# Autodesk Inventor assembly: Chain Testing 9-16-19
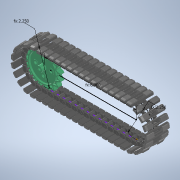
[picture p0: Inventor's stored thumbnail of the model, 180x180]
Saved by Autodesk Inventor 2020 (Build 240168000, 168)
## iProperties
Created: 2019-09-16
Part Number: Chain Testing 9-16-19
Document SubType Name: Assembly
Designer: Corey
Author: Corey
## Documents named in this file (4)
- C:\Users\Corey\Documents\Tower-Takeover-CAD\Chain Testing 9-16-19.iam
- C:\Users\Corey\Documents\Tower-Takeover-CAD\Parts\Motion\Chain & Tank Tread\Tank Tread Traction Link.ipt
- C:\Users\Corey\Documents\Tower-Takeover-CAD\Chain Sketch 9-16-9.ipt
- C:\Users\Corey\Documents\Tower-Takeover-CAD\Parts\Motion\Sprockets\High Strength 18-tooth Sprocket.ipt
## Components (51 placed, 3 different names)
1. Chain Sketch 9-16-9:1 — Flush:1, Flush:2, Flush:3, Flush:4, Flush:5, Flush:6
2. High Strength 18-tooth Sprocket:1 — Flush:4, Flush:5, Flush:6
3. Tank Tread Traction Link:1 — Flush:1, Flush:2, Flush:3
4. Tank Tread Traction Link:2
5. Tank Tread Traction Link:3
6. Tank Tread Traction Link:4
7. Tank Tread Traction Link:5
8. Tank Tread Traction Link:6
9. Tank Tread Traction Link:7
10. Tank Tread Traction Link:8
11. Tank Tread Traction Link:9
12. Tank Tread Traction Link:10
13. Tank Tread Traction Link:11
14. Tank Tread Traction Link:12
15. Tank Tread Traction Link:13
16. Tank Tread Traction Link:14
17. Tank Tread Traction Link:15
18. Tank Tread Traction Link:16
19. Tank Tread Traction Link:17
20. Tank Tread Traction Link:18
21. Tank Tread Traction Link:19
22. Tank Tread Traction Link:20
23. Tank Tread Traction Link:21
24. Tank Tread Traction Link:22
25. Tank Tread Traction Link:23
26. Tank Tread Traction Link:24
27. Tank Tread Traction Link:25
28. Tank Tread Traction Link:26
29. Tank Tread Traction Link:27
30. Tank Tread Traction Link:28
31. Tank Tread Traction Link:29
32. Tank Tread Traction Link:30
33. Tank Tread Traction Link:31
34. Tank Tread Traction Link:32
35. Tank Tread Traction Link:33
36. Tank Tread Traction Link:34
37. Tank Tread Traction Link:35
38. Tank Tread Traction Link:36
39. Tank Tread Traction Link:37
40. Tank Tread Traction Link:38
41. Tank Tread Traction Link:39
42. Tank Tread Traction Link:40
43. Tank Tread Traction Link:41
44. Tank Tread Traction Link:42
45. Tank Tread Traction Link:43
46. Tank Tread Traction Link:44
47. Tank Tread Traction Link:45
48. Tank Tread Traction Link:46
49. Tank Tread Traction Link:47
50. Tank Tread Traction Link:48
51. Tank Tread Traction Link:49
## Component patterns: (49 elements, first: Tank Tread Traction Link:1)
## Relationships (6: Flush 6)
- Flush:1: Chain Sketch 9-16-9:1 ↔ Tank Tread Traction Link:1
- Flush:2 (33.02 mm): Chain Sketch 9-16-9:1 ↔ Tank Tread Traction Link:1
- Flush:3 (-152.4 mm): Chain Sketch 9-16-9:1 ↔ Tank Tread Traction Link:1
- Flush:4: Chain Sketch 9-16-9:1 ↔ High Strength 18-tooth Sprocket:1
- Flush:5: Chain Sketch 9-16-9:1 ↔ High Strength 18-tooth Sprocket:1
- Flush:6: Chain Sketch 9-16-9:1 ↔ High Strength 18-tooth Sprocket:1
